# Autodesk Inventor assembly: service_design_project_draft
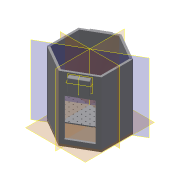
[picture p0: Inventor's stored thumbnail of the model, 180x180]
Saved by Autodesk Inventor 2017 (Build 210142000, 142)
## iProperties
Created: 2018-11-28
Part Number: service_design_project_draft
Document SubType Name: Assembly
Designer: jpb34
Author: jpb34
## Documents named in this file (8)
- C:\Users\jacob\Desktop\service_design_project_draft.iam
- C:\Users\jacob\Desktop\HEX_BASE.ipt
- C:\Users\jacob\Desktop\side.ipt
- C:\Users\jacob\Desktop\Mid_Plate.ipt
- C:\Users\jacob\Desktop\side_w_door.ipt
- C:\Users\jacob\Desktop\handle.ipt
- C:\Users\jacob\Desktop\handle_MIR.ipt
- C:\Users\jacob\Desktop\mid_plate_support.ipt
## Components (13 placed, 7 different names)
1. HEX_BASE:1 — Mate:1, Flush:1, Mate:2, Mate:5, Mate:8, Mate:12
2. Mid_Plate:1 — Mate:5, Mate:6
3. side_w_door:1 — Mate:7, Mate:8, Mate:9, Mate:10, Symmetry:2, Mate:11
4. handle:1 — Mate:9, Mate:10
5. handle_MIR:1
6. side:1 — Mate:1, Flush:1, Mate:2, Symmetry:1, Symmetry:2
7. side:2
8. side:3
9. side:4 — Mate:7
10. side:5 — Mate:6
11. mid_plate_support:3 — Mate:11, Mate:12
12. mid_plate_support:4
13. mid_plate_support:5
## Component patterns: (5 elements, first: side:1), (3 elements, first: mid_plate_support:3)
## Relationships (15: Mate 12, Symmetry 2, Flush 1)
- Mate:1: HEX_BASE:1 ↔ side:1
- Flush:1: HEX_BASE:1 ↔ side:1
- Mate:2: HEX_BASE:1 ↔ side:1
- Symmetry:1: side:1
- Mate:3
- Mate:4
- Mate:5 (101.6 mm): HEX_BASE:1 ↔ Mid_Plate:1
- Mate:6: Mid_Plate:1 ↔ side:5
- Mate:7: side_w_door:1 ↔ side:4
- Mate:8: HEX_BASE:1 ↔ side_w_door:1
- Mate:9 (114.3 mm): side_w_door:1 ↔ handle:1
- Mate:10 (146.05 mm): side_w_door:1 ↔ handle:1
- Symmetry:2: side_w_door:1 ↔ side:1
- Mate:11 (44.45 mm): side_w_door:1 ↔ mid_plate_support:3
- Mate:12 (25.4 mm): HEX_BASE:1 ↔ mid_plate_support:3
